# Autodesk Inventor assembly: DC6V9RPMJGB37-520
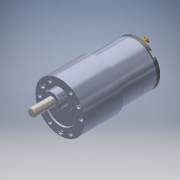
[picture p0: Inventor's stored thumbnail of the model, 180x180]
Saved by Autodesk Inventor 2019 (Build 230136000, 136)
## iProperties
Created: 2017-03-25
Part Number: DC6V9RPMJGB37-520
Document SubType Name: Assembly
Designer: 19879326
Sending System: SolidWorks 2017
Last Author: 1
Last Saved: 2017-12-18
Author: 19879326
## Documents named in this file (9)
- H:\Skripsie\CAD\DC motor\DC_Motor.iam
- H:\Skripsie\CAD\DC motor\JGB37-520_DC6V9RPM\DC6V9RPMGEARED BODY, MOTOR, JGB37-520.ipt
- H:\Skripsie\CAD\DC motor\JGB37-520_DC6V9RPM\DC6V9RPMDC MOTOR, JGB37-520.ipt
- H:\Skripsie\CAD\DC motor\JGB37-520_DC6V9RPM\DC6V9RPMMOTOR SHAFT, JGB37-520.ipt
- H:\Skripsie\CAD\DC motor\JGB37-520_DC6V9RPM\DC6V9RPMSHAFT COUPLER, JGB37-520.ipt
- H:\Skripsie\CAD\DC motor\JGB37-520_DC6V9RPM\DC6V9RPMCOUPLING BRACKET, GEARED BODY TO DC MOTOR, JGB37-520.ipt
- H:\Skripsie\CAD\DC motor\JGB37-520_DC6V9RPM\DC6V9RPMPLASTIC COVER, DC MOTOR, JGB37-520.ipt
- H:\Skripsie\CAD\DC motor\JGB37-520_DC6V9RPM\DC6V9RPMCONNECTION, DC MOTOR, JGB37-520.ipt
- H:\Skripsie\CAD\DC motor\JGB37-520_DC6V9RPM\Деталь2^JGB37-520.ipt
## Components (9 placed, 8 different names)
1. DC6V9RPMGEARED BODY, MOTOR, JGB37-520:1
2. DC6V9RPMDC MOTOR, JGB37-520:1 — Mate:1, Mate:2
3. DC6V9RPMMOTOR SHAFT, JGB37-520:1
4. DC6V9RPMSHAFT COUPLER, JGB37-520:1
5. DC6V9RPMCOUPLING BRACKET, GEARED BODY TO DC MOTOR, JGB37-520:1
6. DC6V9RPMPLASTIC COVER, DC MOTOR, JGB37-520:1 — Mate:1, Mate:2, Mate:3, Mate:4, Mate:5, Mate:6
7. DC6V9RPMCONNECTION, DC MOTOR, JGB37-520:1 — Mate:4, Mate:5
8. DC6V9RPMCONNECTION, DC MOTOR, JGB37-520:2 — Mate:3, Mate:6
9. Деталь2^JGB37-520:1
## Relationships (6: Mate 6)
- Mate:1: DC6V9RPMDC MOTOR, JGB37-520:1 ↔ DC6V9RPMPLASTIC COVER, DC MOTOR, JGB37-520:1
- Mate:2: DC6V9RPMDC MOTOR, JGB37-520:1 ↔ DC6V9RPMPLASTIC COVER, DC MOTOR, JGB37-520:1
- Mate:3: DC6V9RPMPLASTIC COVER, DC MOTOR, JGB37-520:1 ↔ DC6V9RPMCONNECTION, DC MOTOR, JGB37-520:2
- Mate:4: DC6V9RPMPLASTIC COVER, DC MOTOR, JGB37-520:1 ↔ DC6V9RPMCONNECTION, DC MOTOR, JGB37-520:1
- Mate:5: DC6V9RPMPLASTIC COVER, DC MOTOR, JGB37-520:1 ↔ DC6V9RPMCONNECTION, DC MOTOR, JGB37-520:1
- Mate:6: DC6V9RPMPLASTIC COVER, DC MOTOR, JGB37-520:1 ↔ DC6V9RPMCONNECTION, DC MOTOR, JGB37-520:2
